# Autodesk Inventor assembly: BumberAssembly.ver1-1111-2020
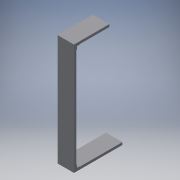
[picture p0: Inventor's stored thumbnail of the model, 180x180]
Saved by Autodesk Inventor 2018 (Build 220112000, 112)
## iProperties
Created: 2020-01-28
Part Number: BumberAssembly.ver1-1111-2020
Document SubType Name: Assembly
Designer: JMHal
Author: JMHal
## Documents named in this file (5)
- F:\GrabCad\2020 Infinite Recharge\BumberAssembly.ver1-1111-2020.iam
- F:\GrabCad\2020 Infinite Recharge\BumberSide.ver1-1111-2020.ipt
- F:\GrabCad\2020 Infinite Recharge\BumberFront.ver1-1111-2020.ipt
- F:\GrabCad\2020 Infinite Recharge\BumberBack.ver1-1111-2020.ipt
- F:\GrabCad\2020 Infinite Recharge\BumberGusset.ver1-1111-2020.ipt
## Components (5 placed, 4 different names)
1. BumberSide.ver1-1111-2020:1 — Flush:2, Mate:1, Flush:3, Mate:2, Flush:4, Flush:5, Mate:4, Mate:6, Flush:7
2. BumberFront.ver1-1111-2020:1 — Mate:2, Flush:4, Flush:5, Mate:3, Flush:6
3. BumberBack.ver1-1111-2020:1 — Flush:2, Mate:1, Flush:3, Mate:5
4. BumberGusset.ver1-1111-2020:1 — Mate:3, Mate:4, Flush:6
5. BumberGusset.ver1-1111-2020:2 — Mate:5, Mate:6, Flush:7
## Relationships (12: Flush 6, Mate 6)
- Flush:2: BumberSide.ver1-1111-2020:1 ↔ BumberBack.ver1-1111-2020:1
- Mate:1: BumberSide.ver1-1111-2020:1 ↔ BumberBack.ver1-1111-2020:1
- Flush:3: BumberSide.ver1-1111-2020:1 ↔ BumberBack.ver1-1111-2020:1
- Mate:2: BumberSide.ver1-1111-2020:1 ↔ BumberFront.ver1-1111-2020:1
- Flush:4: BumberSide.ver1-1111-2020:1 ↔ BumberFront.ver1-1111-2020:1
- Flush:5: BumberSide.ver1-1111-2020:1 ↔ BumberFront.ver1-1111-2020:1
- Mate:3: BumberFront.ver1-1111-2020:1 ↔ BumberGusset.ver1-1111-2020:1
- Mate:4: BumberSide.ver1-1111-2020:1 ↔ BumberGusset.ver1-1111-2020:1
- Flush:6: BumberFront.ver1-1111-2020:1 ↔ BumberGusset.ver1-1111-2020:1
- Mate:5: BumberBack.ver1-1111-2020:1 ↔ BumberGusset.ver1-1111-2020:2
- Mate:6: BumberSide.ver1-1111-2020:1 ↔ BumberGusset.ver1-1111-2020:2
- Flush:7: BumberSide.ver1-1111-2020:1 ↔ BumberGusset.ver1-1111-2020:2
